# Autodesk Inventor assembly: frame assy
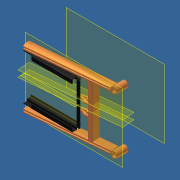
[picture p0: Inventor's stored thumbnail of the model, 180x180]
Saved by Autodesk Inventor 2012 (Build 160160000, 160)
## iProperties
Created: 2012-03-07
Part Number: frame assy
Document SubType Name: Assembly
Designer: esv
Mass: 22101.3 g
Surface Area: 8904.59 cm^2
Volume: 6785.47 cm^3
Density: 3.25715 g/cm^3
Author: esv
## Documents named in this file (3)
- C:\Users\Edward\Documents\masters\CAD\Invacare\frame assy.iam
- C:\Users\Edward\Documents\masters\CAD\Invacare\frame.ipt
- C:\Users\Edward\Documents\masters\CAD\Invacare\battery rails.ipt
## Components (2 placed, 2 different names)
1. frame:1 — Angle:2, Mate:9, Flush:10, Angle:3
2. battery rails:1 — Mate:7, Flush:3, Mate:9, Flush:10
## Relationships (6: Mate 2, Flush 2, Angle 2)
- Mate:7: battery rails:1
- Flush:3: battery rails:1
- Angle:2 (0 deg): frame:1
- Mate:9: frame:1 ↔ battery rails:1
- Flush:10: frame:1 ↔ battery rails:1
- Angle:3 (0 deg): frame:1
